# Autodesk Inventor assembly: front_panel
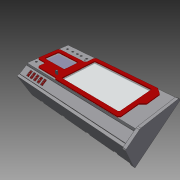
[picture p0: Inventor's stored thumbnail of the model, 180x180]
Saved by Autodesk Inventor 2014 (Build 180170000, 170)
## iProperties
Created: 2014-03-22
Part Number: front_panel
Document SubType Name: Assembly
Designer: buben
Author: buben
## Documents named in this file (13)
- C:\Users\buben\Documents\GitHub\bacon\inventor files\printer parts\6.5 mm\front_panel.iam
- C:\Users\buben\Documents\GitHub\bacon\inventor files\printer parts\6.5 mm\main_lcd_front.ipt
- C:\Users\buben\Documents\GitHub\bacon\inventor files\utils\controller_lcd_cover_glass.ipt
- C:\Users\buben\Documents\GitHub\bacon\inventor files\utils\main_lcd_cover_glass.ipt
- C:\Users\buben\Documents\GitHub\bacon\inventor files\utils\main_lcd_panel.ipt
- C:\Users\buben\Documents\GitHub\bacon\inventor files\utils\ramps_smart_controller\controler.iam
- C:\Users\buben\Documents\GitHub\bacon\inventor files\utils\main_lcd_controller\lcd_controller.iam
- C:\Users\buben\Documents\GitHub\bacon\inventor files\printer parts\6.5 mm\front_panel_brace_right.ipt
- C:\Users\buben\Documents\GitHub\bacon\inventor files\printer parts\6.5 mm\front_panel_middle.ipt
- C:\Users\buben\Documents\GitHub\bacon\inventor files\printer parts\6.5 mm\front_panel_bottom.ipt
- C:\Users\buben\Documents\GitHub\bacon\inventor files\3rd party components\USB socket\Imported Components\USB-Socket\USB-Socket.ipt
- C:\Users\buben\Documents\GitHub\bacon\inventor files\printer parts\6.5 mm\front_panel_brace_middle.ipt
- C:\Users\buben\Documents\GitHub\bacon\inventor files\utils\front_panel_frame.ipt
## Components (16 placed, 12 different names)
1. main_lcd_front:1 — Mate:1, Mate:2, Mate:3, Flush:1, Flush:2, Mate:4, Mate:5, Mate:6, Mate:7, Mate:9, Mate:10, Mate:12, Mate:13, Mate:14, Angle:1, Mate:15, Mate:16, Flush:3, Mate:19, Mate:28, Mate:29, Mate:30
2. controller_lcd_cover_glass:1 — Flush:2, Mate:6, Mate:7, Mate:11
3. main_lcd_cover_glass:1 — Flush:1, Mate:4, Mate:5, Mate:8
4. main_lcd_panel:1 — Mate:8, Mate:9, Mate:10
5. controler:1 [sub-assembly] — Mate:11, Mate:12, Mate:13, Mate:27
6. lcd_controller:1 [sub-assembly] — Mate:14, Angle:1, Mate:15
7. front_panel_brace_right:1 — Mate:16, Flush:3, Mate:17, Flush:4, Mate:18, Flush:5, Mate:21
8. front_panel_middle:1 — Mate:17, Flush:4, Mate:19, Mate:20, Mate:22, Mate:23, Mate:24, Mate:26
9. front_panel_bottom:1 — Mate:18, Flush:5, Mate:20, Mate:21, Mate:25
10. front_panel_brace_middle:1 — Mate:25, Mate:26, Mate:27
11. front_panel_frame:1 — Mate:28, Mate:29, Mate:30
12. USB-Socket:1 — Mate:22, Mate:23, Mate:24
13. USB-Socket:2
14. USB-Socket:3
15. USB-Socket:4
16. USB-Socket:5
## Component patterns: (5 elements, first: USB-Socket:1)
## Relationships (36: Mate 30, Flush 5, Angle 1)
- Mate:1: main_lcd_front:1
- Mate:2: main_lcd_front:1
- Mate:3: main_lcd_front:1
- Flush:1: main_lcd_front:1 ↔ main_lcd_cover_glass:1
- Flush:2: main_lcd_front:1 ↔ controller_lcd_cover_glass:1
- Mate:4: main_lcd_front:1 ↔ main_lcd_cover_glass:1
- Mate:5 (0.5 mm): main_lcd_front:1 ↔ main_lcd_cover_glass:1
- Mate:6: main_lcd_front:1 ↔ controller_lcd_cover_glass:1
- Mate:7: main_lcd_front:1 ↔ controller_lcd_cover_glass:1
- Mate:8 (0.5 mm): main_lcd_cover_glass:1 ↔ main_lcd_panel:1
- Mate:9: main_lcd_front:1 ↔ main_lcd_panel:1
- Mate:10: main_lcd_front:1 ↔ main_lcd_panel:1
- Mate:11: controller_lcd_cover_glass:1 ↔ controler:1
- Mate:12 (0.9 mm): main_lcd_front:1 ↔ controler:1
- Mate:13 (-0.5 mm): main_lcd_front:1 ↔ controler:1
- Mate:14: main_lcd_front:1 ↔ lcd_controller:1
- Angle:1 (0 deg): main_lcd_front:1 ↔ lcd_controller:1
- Mate:15 (5 mm): main_lcd_front:1 ↔ lcd_controller:1
- Mate:16: main_lcd_front:1 ↔ front_panel_brace_right:1
- Flush:3 (3 mm): main_lcd_front:1 ↔ front_panel_brace_right:1
- Mate:17: front_panel_brace_right:1 ↔ front_panel_middle:1
- Flush:4 (3 mm): front_panel_brace_right:1 ↔ front_panel_middle:1
- Mate:18: front_panel_brace_right:1 ↔ front_panel_bottom:1
- Flush:5 (3 mm): front_panel_brace_right:1 ↔ front_panel_bottom:1
- Mate:19 (1 mm): main_lcd_front:1 ↔ front_panel_middle:1
- Mate:20 (1 mm): front_panel_middle:1 ↔ front_panel_bottom:1
- Mate:21 (-1 mm): front_panel_brace_right:1 ↔ front_panel_bottom:1
- Mate:22: front_panel_middle:1 ↔ USB-Socket:1
- Mate:23 (0.5 mm): front_panel_middle:1 ↔ USB-Socket:1
- Mate:24 (0.5 mm): front_panel_middle:1 ↔ USB-Socket:1
- Mate:25: front_panel_bottom:1 ↔ front_panel_brace_middle:1
- Mate:26: front_panel_middle:1 ↔ front_panel_brace_middle:1
- Mate:27: controler:1 ↔ front_panel_brace_middle:1
- Mate:28: main_lcd_front:1 ↔ front_panel_frame:1
- Mate:29 (-5 mm): main_lcd_front:1 ↔ front_panel_frame:1
- Mate:30 (-5 mm): main_lcd_front:1 ↔ front_panel_frame:1
